# Autodesk Inventor assembly: gakutasu-cat-wheel
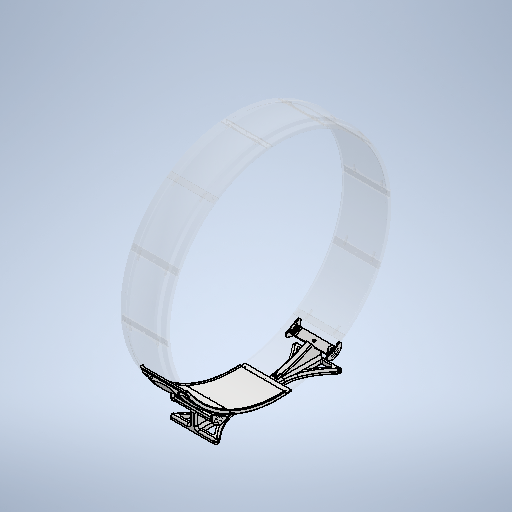
[picture p0: Inventor's stored thumbnail of the model, 512x512]
Saved by Autodesk Inventor 2026.3 (Build 303398000, 398)
## iProperties
Created: 2026-01-17
Part Number: gakutasu-cat-wheel
Document SubType Name: Assembly
Designer: gakut
Author: gakut
## Documents named in this file (8)
- C:\Users\gakut\Documents\Inventor\gakutasu-cat-wheel\gakutasu-cat-wheel.iam
- C:\Users\gakut\Documents\Inventor\gakutasu-cat-wheel\parts\wheel_plate.ipt
- C:\Users\gakut\Documents\Inventor\gakutasu-cat-wheel\parts\plate_joint_shaft.ipt
- C:\Users\gakut\Documents\Inventor\gakutasu-cat-wheel\parts\caster_d25.ipt
- C:\Users\gakut\Documents\Inventor\gakutasu-cat-wheel\parts\caster_holder.ipt
- C:\Users\gakut\Documents\Inventor\gakutasu-cat-wheel\parts\base_center.ipt
- C:\Users\gakut\Documents\Inventor\gakutasu-cat-wheel\parts\base_side.ipt
- C:\Users\gakut\Documents\Inventor\gakutasu-cat-wheel\parts\base_cover.ipt
## Components (26 placed, 7 different names)
1. wheel_plate:1 — Mate:1, Flush:1, Mate:2, Mate:3, Flush:7, Tangent:3
2. plate_joint_shaft:1 — Mate:1, Flush:1
3. wheel_plate:2 — Mate:2, Mate:3, Mate:6, Mate:7
4. wheel_plate:3 — Mate:6, Mate:7
5. wheel_plate:4 — Mate:14, Mate:15
6. wheel_plate:5 — Mate:14, Mate:15
7. wheel_plate:6
8. wheel_plate:7
9. wheel_plate:8 — Mate:22, Mate:23
10. wheel_plate:9 — Mate:22, Mate:23
11. wheel_plate:10
12. wheel_plate:11 — Tangent:2
13. wheel_plate:12
14. caster_d25:1 — Insert:1, Insert:2, Tangent:3
15. caster_holder:1 — Insert:1, Insert:2, Insert:3, Insert:4, Mate:25, Insert:12, Insert:14, Flush:8, Insert:15, Flush:9
16. caster_d25:2 — Insert:3, Insert:4
17. base_center:1 — Flush:2, Flush:3, Mate:24, Mate:27, Insert:11, Flush:4, Flush:5, Flush:6
18. base_side:1 — Flush:2, Flush:3, Mate:24, Mate:25, Insert:12
19. caster_d25:3
20. caster_holder:2 — Insert:13, Insert:16, Flush:10, Insert:17, Flush:11
21. caster_d25:4 — Tangent:2
22. base_side:2 — Mate:27, Insert:11, Insert:13
23. base_cover:1 — Insert:14, Flush:8
24. base_cover:2 — Insert:15, Flush:9
25. base_cover:3 — Insert:17, Flush:11
26. base_cover:4 — Insert:16, Flush:10
## Relationships (55: Mate 27, Insert 15, Flush 11, Tangent 2)
- Mate:1: wheel_plate:1 ↔ plate_joint_shaft:1
- Flush:1: wheel_plate:1 ↔ plate_joint_shaft:1
- Mate:2: wheel_plate:1 ↔ wheel_plate:2
- Mate:3: wheel_plate:1 ↔ wheel_plate:2
- [Mate]: wheel_plate:3 ↔ wheel_plate:4
- [Mate]: wheel_plate:3 ↔ wheel_plate:4
- Mate:6: wheel_plate:2 ↔ wheel_plate:3
- Mate:7: wheel_plate:2 ↔ wheel_plate:3
- [Mate]: wheel_plate:5 ↔ wheel_plate:6
- [Mate]: wheel_plate:5 ↔ wheel_plate:6
- [Mate]: wheel_plate:7 ↔ wheel_plate:8
- [Mate]: wheel_plate:7 ↔ wheel_plate:8
- [Mate]: wheel_plate:6 ↔ wheel_plate:7
- [Mate]: wheel_plate:6 ↔ wheel_plate:7
- Mate:14: wheel_plate:4 ↔ wheel_plate:5
- Mate:15: wheel_plate:4 ↔ wheel_plate:5
- [Mate]: wheel_plate:9 ↔ wheel_plate:10
- [Mate]: wheel_plate:9 ↔ wheel_plate:10
- [Mate]: wheel_plate:11 ↔ wheel_plate:12
- [Mate]: wheel_plate:11 ↔ wheel_plate:12
- [Mate]: wheel_plate:10 ↔ wheel_plate:11
- [Mate]: wheel_plate:10 ↔ wheel_plate:11
- Mate:22: wheel_plate:8 ↔ wheel_plate:9
- Mate:23: wheel_plate:8 ↔ wheel_plate:9
- Insert:1: caster_d25:1 ↔ caster_holder:1
- Insert:2: caster_d25:1 ↔ caster_holder:1
- Insert:3: caster_holder:1 ↔ caster_d25:2
- Insert:4: caster_holder:1 ↔ caster_d25:2
- Flush:2: base_center:1 ↔ base_side:1
- Flush:3: base_center:1 ↔ base_side:1
- Mate:24: base_center:1 ↔ base_side:1
- Mate:25: caster_holder:1 ↔ base_side:1
- [Insert]: caster_d25:3 ↔ caster_holder:2
- [Insert]: caster_d25:3 ↔ caster_holder:2
- [Insert]: caster_holder:2 ↔ caster_d25:4
- [Insert]: caster_holder:2 ↔ caster_d25:4
- [Mate]: caster_holder:2 ↔ base_side:2
- Mate:27: base_center:1 ↔ base_side:2
- Insert:11: base_center:1 ↔ base_side:2
- Flush:4: base_center:1
- Flush:5: base_center:1
- Flush:6: base_center:1
- Flush:7: wheel_plate:1
- Insert:12: caster_holder:1 ↔ base_side:1
- Insert:13: caster_holder:2 ↔ base_side:2
- Insert:14: caster_holder:1 ↔ base_cover:1
- Flush:8: caster_holder:1 ↔ base_cover:1
- Insert:15: caster_holder:1 ↔ base_cover:2
- Flush:9: caster_holder:1 ↔ base_cover:2
- Insert:16: caster_holder:2 ↔ base_cover:4
- Flush:10: caster_holder:2 ↔ base_cover:4
- Insert:17: caster_holder:2 ↔ base_cover:3
- Flush:11: caster_holder:2 ↔ base_cover:3
- Tangent:2: wheel_plate:11 ↔ caster_d25:4
- Tangent:3: wheel_plate:1 ↔ caster_d25:1
## Named parameters: d32_d30 = 0 mm, d33_d31 = 0 mm, d36_d30 = 0 mm, d37_d31 = 0 mm, d38_d32_d30 = 0 mm, d39_d33_d31 = 0 mm, d40_d34 = 0 mm, d41_d35 = 0 mm, d44_d30 = 0 mm, d45_d31 = 0 mm, d46_d32_d30 = 0 mm, d47_d33_d31 = 0 mm, d48_d34 = 0 mm, d49_d35 = 0 mm, d62_d52 = 0 mm, d63_d53 = 0 mm, d64_d54 = 0 mm, d65_d55 = 0 mm, d66_d60 = 0 mm
